# Autodesk Inventor assembly: Robot Inesco
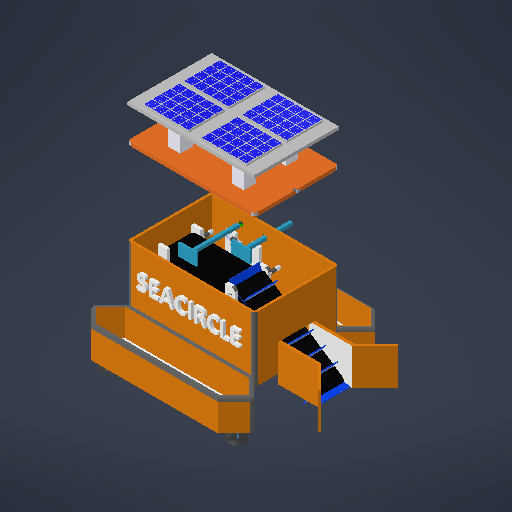
[picture p0: Inventor's stored thumbnail of the model, 512x512]
Saved by Autodesk Inventor 2026.2 (Build 302298000, 298)
## iProperties
Created: 2025-12-05
Part Number: Robot Inesco
Document SubType Name: Assembly
Designer: hando
Author: hando
## Documents named in this file (16)
- D:\Data_Lokal\Kuliah\Tri Wahyu (22518241023)\Lomba Essay\INESCO 2025\Robot Inesco.iam
- D:\Data_Lokal\Kuliah\Tri Wahyu (22518241023)\Lomba Essay\Himpunan Administrasi Publik UNY\Design Kapal\Solar panel.ipt
- D:\Data_Lokal\Kuliah\Tri Wahyu (22518241023)\Lomba Essay\INESCO 2025\Base iNESCO.ipt
- D:\Data_Lokal\Kuliah\Tri Wahyu (22518241023)\Lomba Essay\INESCO 2025\Wadah 45l.ipt
- D:\Data_Lokal\Kuliah\Tri Wahyu (22518241023)\Lomba Essay\INESCO 2025\Belt Angkut.ipt
- D:\Data_Lokal\Kuliah\Tri Wahyu (22518241023)\Lomba Essay\INESCO 2025\Belt Pilah.ipt
- D:\Data_Lokal\Kuliah\Tri Wahyu (22518241023)\Lomba Essay\INESCO 2025\T500-THRUSTER-R1.ipt
- D:\Data_Lokal\Kuliah\Tri Wahyu (22518241023)\Lomba Essay\INESCO 2025\dc-motor-24v-pg-56-19-2k-13ppr-brake-1.snapshot.2\DC Motor 24V PG 56 19.2K 13PPR Brake\DC Motor 24V PG 56 19.2K 13PPR Brake\DC Motor 24V PG 5.ipt
- D:\Data_Lokal\Kuliah\Tri Wahyu (22518241023)\Lomba Essay\INESCO 2025\Linear Actuator.ipt
- D:\Data_Lokal\Kuliah\Tri Wahyu (22518241023)\Lomba Essay\INESCO 2025\Tutup Atas.ipt
- D:\Data_Lokal\Kuliah\Tri Wahyu (22518241023)\Lomba Essay\Himpunan Administrasi Publik UNY\Design Kapal\BATERIA.ipt
- D:\Data_Lokal\Kuliah\Tri Wahyu (22518241023)\Lomba Essay\INESCO 2025\driverbtn v1.iam
- D:\Data_Lokal\Kuliah\Tri Wahyu (22518241023)\Lomba Essay\Himpunan Administrasi Publik UNY\Design Kapal\raspberry-pi-5-2.snapshot.8\RASPBERRY_PI_5\RASPBERRY_PI_5\RASPBERRY_PI_5.iam
- D:\Data_Lokal\Kuliah\Tri Wahyu (22518241023)\Lomba Essay\INESCO 2025\Logitech c270 Assembly.iam
- D:\Data_Lokal\Kuliah\Tri Wahyu (22518241023)\Lomba Essay\Himpunan Administrasi Publik UNY\Design Kapal\ph-sensor-1.snapshot.1\pH_Sensor\pH_Sensor\pH_Sensor.iam
- D:\Data_Lokal\Kuliah\Tri Wahyu (22518241023)\Lomba Essay\Himpunan Administrasi Publik UNY\Design Kapal\dfrobot-gravity-dissolved-oxygen-sensor-v1-0-1.snapshot.1\Gravity Dissolved Oxygen Sensor v1.0\Gravity Diss.ipt
## Components (33 placed, 15 different names)
1. Tutup Atas:1 — Mate:40, Mate:41, Mate:42, Mate:43, Mate:44, Mate:45, Flush:2, Flush:3, Flush:4, Flush:5, Flush:6, Flush:7, Flush:8, Flush:9, Mate:48, Mate:51, Mate:56, Mate:57, Mate:58, Mate:59, Mate:60, Flush:14, Mate:62, Flush:15, Mate:63, Flush:16, Mate:65, Flush:18, Flush:19, Mate:66, Mate:67, Mate:69
2. Solar panel:3 — Mate:45, Flush:4, Flush:5
3. Solar panel:4 — Mate:43, Flush:2, Flush:3
4. Logitech c270 Assembly:1 [sub-assembly] — Mate:65, Flush:18, Flush:19
5. driverbtn v1:8 [sub-assembly] — Mate:66, Mate:67, Flush:20, Mate:68, Mate:70, Flush:21
6. driverbtn v1:7 [sub-assembly] — Mate:68, Mate:69, Flush:21
7. driverbtn v1:2 [sub-assembly] — Mate:55, Flush:13, Mate:59, Flush:20, Mate:70
8. RASPBERRY_PI_5:1 [sub-assembly] — Mate:62, Flush:15, Mate:63
9. Solar panel:1 — Mate:42, Flush:6, Flush:7
10. Solar panel:2 — Mate:44, Flush:8, Flush:9
11. driverbtn v1:4 [sub-assembly] — Mate:54, Mate:55, Flush:12, Flush:13, Mate:58
12. driverbtn v1:3 [sub-assembly] — Mate:53, Mate:54, Flush:11, Flush:12, Mate:60, Mate:61
13. driverbtn v1:5 [sub-assembly] — Mate:52, Flush:10, Mate:57, Mate:64, Flush:17
14. driverbtn v1:6 [sub-assembly] — Mate:52, Mate:53, Flush:10, Flush:11, Mate:56, Mate:61, Flush:14
15. driverbtn v1:1 [sub-assembly] — Mate:51, Mate:64, Flush:17
16. BATERIA:1 — Mate:48, Flush:16
17. Base iNESCO:1 — Mate:1, Mate:2, Mate:3, Mate:4, Mate:5, Mate:6, Mate:7, Mate:8, Mate:29, Mate:40, Mate:41, Mate:46, Mate:47, Mate:71, Mate:72, Mate:73, Mate:74, Mate:75, Mate:76, Mate:77, Mate:78, Mate:79, Mate:80, Mate:82, Mate:83, Mate:84, Mate:85, Mate:86
18. Wadah 45l:1 — Mate:1, Mate:2, Mate:28, Mate:29, Mate:30
19. Wadah 45l:2 — Mate:3, Mate:4, Mate:30, Mate:32
20. Belt Angkut:1 — Mate:5, Mate:6
21. Belt Pilah:1 — Mate:7, Mate:8, Mate:35, Mate:37
22. T500-THRUSTER-R1:1 — Mate:71, Mate:72, Mate:73, Mate:74
23. T500-THRUSTER-R1:2 — Mate:78, Mate:79, Mate:80
24. T500-THRUSTER-R1:3 — Mate:82, Mate:83, Mate:84
25. T500-THRUSTER-R1:4 — Mate:75, Mate:76, Mate:77
26. DC Motor 24V PG 5:1 — Flush:1, Mate:39
27. Linear Actuator:1 — Mate:28, Flush:1, Mate:35, Mate:39
28. Linear Actuator:2 — Mate:32, Mate:36, Mate:37, Mate:38
29. DC Motor 24V PG 5:2 — Mate:36, Mate:38
30. DC Motor 24V PG 5:3 — Mate:46
31. DC Motor 24V PG 5:4 — Mate:47
32. pH_Sensor:1 [sub-assembly] — Mate:85
33. Gravity Diss:1 — Mate:86
## Relationships (82: Mate 61, Flush 21)
- Mate:1: Base iNESCO:1 ↔ Wadah 45l:1
- Mate:2: Base iNESCO:1 ↔ Wadah 45l:1
- Mate:3: Base iNESCO:1 ↔ Wadah 45l:2
- Mate:4: Base iNESCO:1 ↔ Wadah 45l:2
- Mate:5: Base iNESCO:1 ↔ Belt Angkut:1
- Mate:6: Base iNESCO:1 ↔ Belt Angkut:1
- Mate:7: Base iNESCO:1 ↔ Belt Pilah:1
- Mate:8: Base iNESCO:1 ↔ Belt Pilah:1
- Mate:28: Wadah 45l:1 ↔ Linear Actuator:1
- Mate:29 (950 mm): Base iNESCO:1 ↔ Wadah 45l:1
- Mate:30 (50 mm): Wadah 45l:1 ↔ Wadah 45l:2
- Mate:32: Wadah 45l:2 ↔ Linear Actuator:2
- Flush:1 (-10 mm): DC Motor 24V PG 5:1 ↔ Linear Actuator:1
- Mate:35: Belt Pilah:1 ↔ Linear Actuator:1
- Mate:36 (10 mm): Linear Actuator:2 ↔ DC Motor 24V PG 5:2
- Mate:37: Belt Pilah:1 ↔ Linear Actuator:2
- Mate:38: Linear Actuator:2 ↔ DC Motor 24V PG 5:2
- Mate:39: DC Motor 24V PG 5:1 ↔ Linear Actuator:1
- Mate:40: Tutup Atas:1 ↔ Base iNESCO:1
- Mate:41: Tutup Atas:1 ↔ Base iNESCO:1
- Mate:42: Tutup Atas:1 ↔ Solar panel:1
- Mate:43: Tutup Atas:1 ↔ Solar panel:4
- Mate:44: Tutup Atas:1 ↔ Solar panel:2
- Mate:45: Tutup Atas:1 ↔ Solar panel:3
- Flush:2 (60 mm): Tutup Atas:1 ↔ Solar panel:4
- Flush:3 (190 mm): Tutup Atas:1 ↔ Solar panel:4
- Flush:4 (190 mm): Tutup Atas:1 ↔ Solar panel:3
- Flush:5 (60 mm): Tutup Atas:1 ↔ Solar panel:3
- Flush:6 (190 mm): Tutup Atas:1 ↔ Solar panel:1
- Flush:7 (60 mm): Tutup Atas:1 ↔ Solar panel:1
- Flush:8 (190 mm): Tutup Atas:1 ↔ Solar panel:2
- Flush:9 (60 mm): Tutup Atas:1 ↔ Solar panel:2
- Mate:46: Base iNESCO:1 ↔ DC Motor 24V PG 5:3
- Mate:47: Base iNESCO:1 ↔ DC Motor 24V PG 5:4
- Mate:48: Tutup Atas:1 ↔ BATERIA:1
- Mate:51: Tutup Atas:1 ↔ driverbtn v1:1
- Mate:52: driverbtn v1:5 ↔ driverbtn v1:6
- Mate:53: driverbtn v1:3 ↔ driverbtn v1:6
- Mate:54: driverbtn v1:4 ↔ driverbtn v1:3
- Mate:55: driverbtn v1:2 ↔ driverbtn v1:4
- Flush:10: driverbtn v1:5 ↔ driverbtn v1:6
- Flush:11: driverbtn v1:3 ↔ driverbtn v1:6
- Flush:12: driverbtn v1:4 ↔ driverbtn v1:3
- Flush:13: driverbtn v1:2 ↔ driverbtn v1:4
- Mate:56: Tutup Atas:1 ↔ driverbtn v1:6
- Mate:57: Tutup Atas:1 ↔ driverbtn v1:5
- Mate:58: Tutup Atas:1 ↔ driverbtn v1:4
- Mate:59: Tutup Atas:1 ↔ driverbtn v1:2
- Mate:60: Tutup Atas:1 ↔ driverbtn v1:3
- Mate:61: driverbtn v1:3 ↔ driverbtn v1:6
- Flush:14: Tutup Atas:1 ↔ driverbtn v1:6
- Mate:62: Tutup Atas:1 ↔ RASPBERRY_PI_5:1
- Flush:15: Tutup Atas:1 ↔ RASPBERRY_PI_5:1
- Mate:63: Tutup Atas:1 ↔ RASPBERRY_PI_5:1
- Flush:16: Tutup Atas:1 ↔ BATERIA:1
- Mate:64: driverbtn v1:5 ↔ driverbtn v1:1
- Flush:17: driverbtn v1:5 ↔ driverbtn v1:1
- Mate:65: Tutup Atas:1 ↔ Logitech c270 Assembly:1
- Flush:18 (700 mm): Tutup Atas:1 ↔ Logitech c270 Assembly:1
- Flush:19: Tutup Atas:1 ↔ Logitech c270 Assembly:1
- Mate:66: Tutup Atas:1 ↔ driverbtn v1:8
- Mate:67: Tutup Atas:1 ↔ driverbtn v1:8
- Flush:20: driverbtn v1:8 ↔ driverbtn v1:2
- Mate:68: driverbtn v1:8 ↔ driverbtn v1:7
- Mate:69: Tutup Atas:1 ↔ driverbtn v1:7
- Mate:70: driverbtn v1:8 ↔ driverbtn v1:2
- Flush:21: driverbtn v1:8 ↔ driverbtn v1:7
- Mate:71: Base iNESCO:1 ↔ T500-THRUSTER-R1:1
- Mate:72: Base iNESCO:1 ↔ T500-THRUSTER-R1:1
- Mate:73: Base iNESCO:1 ↔ T500-THRUSTER-R1:1
- Mate:74: Base iNESCO:1 ↔ T500-THRUSTER-R1:1
- Mate:75: Base iNESCO:1 ↔ T500-THRUSTER-R1:4
- Mate:76: Base iNESCO:1 ↔ T500-THRUSTER-R1:4
- Mate:77: Base iNESCO:1 ↔ T500-THRUSTER-R1:4
- Mate:78: Base iNESCO:1 ↔ T500-THRUSTER-R1:2
- Mate:79: Base iNESCO:1 ↔ T500-THRUSTER-R1:2
- Mate:80: Base iNESCO:1 ↔ T500-THRUSTER-R1:2
- Mate:82: Base iNESCO:1 ↔ T500-THRUSTER-R1:3
- Mate:83: Base iNESCO:1 ↔ T500-THRUSTER-R1:3
- Mate:84: Base iNESCO:1 ↔ T500-THRUSTER-R1:3
- Mate:85: Base iNESCO:1 ↔ pH_Sensor:1
- Mate:86: Base iNESCO:1 ↔ Gravity Diss:1
